# Autodesk Inventor assembly: ASY Кассета
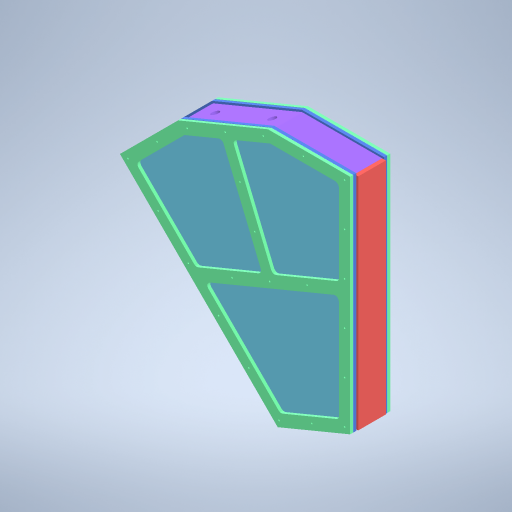
[picture p0: Inventor's stored thumbnail of the model, 512x512]
Saved by Autodesk Inventor 2024.2 (Build 282272000, 272)
## iProperties
Created: 2024-05-05
Part Number: ASY Кассета
Document SubType Name: Assembly
Designer: pokla
Author: pokla
## Documents named in this file (2)
- C:\Users\pokla\Documents\Inventor\ДФО\ДМФ\ДМФ 04.05.24 11-26\ASY ДМФГиД 01011 Кассета.iam
- C:\Users\pokla\Documents\Inventor\ДФО\ДМФ\ДМФ 04.05.24 11-26\ASY Кассета.iam
## Components (1 placed, 1 different names)
1. ASY Кассета:1 [sub-assembly]
## Relationships (1: Mate 1)
- [Mate]: ASY Кассета:1
